# Autodesk Inventor assembly: back lower roller
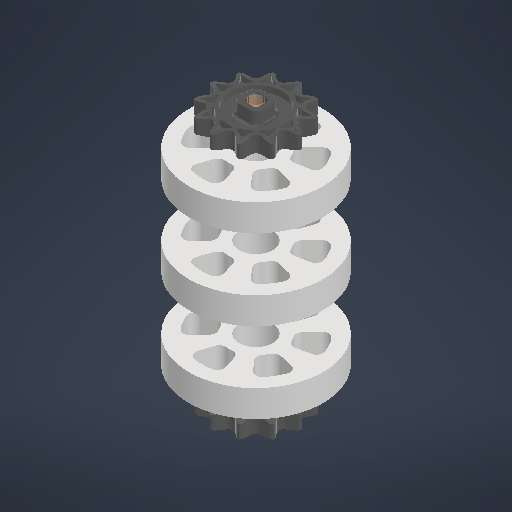
[picture p0: Inventor's stored thumbnail of the model, 512x512]
Saved by Autodesk Inventor 2025.2 (Build 292293000, 293)
## iProperties
Created: 2025-12-04
Part Number: back lower roller
Document SubType Name: Assembly
Designer: cloudy
Author: cloudy
## Documents named in this file (4)
- C:\Users\cloudy\Documents\GitHub\aura-cad\15\back lower roller.iam
- C:\Users\cloudy\Documents\GitHub\aura-cad\15\2.5in flex.ipt
- C:\Users\cloudy\Documents\GitHub\aura-cad\!lib\Motion\Sprockets\9P Sprocket\9P 12T Sprocket, No Insert.iam
- C:\Users\cloudy\Documents\GitHub\aura-cad\!lib\Motion\Sprockets\9P Sprocket.iam
## Components (5 placed, 2 different names)
1. 2.5in flex:1 — Insert:1, Insert:3
2. 2.5in flex:2 — Insert:1, Insert:2, Insert:4
3. 9P 12T Sprocket, No Insert:1 [sub-assembly] — Insert:2
4. 9P 12T Sprocket, No Insert:2 [sub-assembly] — Insert:3
5. 2.5in flex:3 — Insert:4
## Relationships (4: Insert 4)
- Insert:1 (63.5 mm): 2.5in flex:1 ↔ 2.5in flex:2
- Insert:2 (6.35 mm): 2.5in flex:2 ↔ 9P 12T Sprocket, No Insert:1
- Insert:3 (6.35 mm): 2.5in flex:1 ↔ 9P 12T Sprocket, No Insert:2
- Insert:4 (25.4 mm): 2.5in flex:2 ↔ 2.5in flex:3
